# Autodesk Inventor assembly: CONVEYOR-02
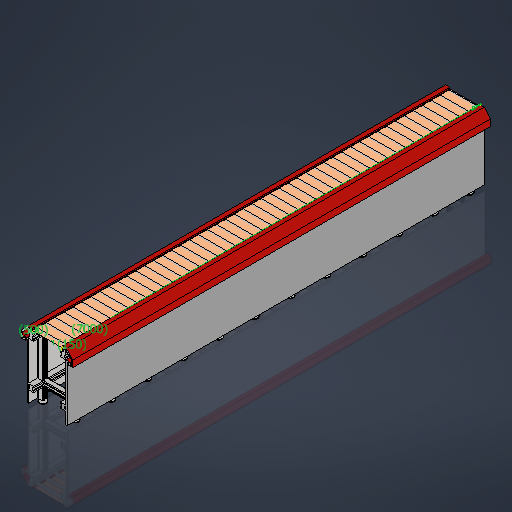
[picture p0: Inventor's stored thumbnail of the model, 512x512]
Saved by Autodesk Inventor 2025 (Build 290162000, 162)
## iProperties
RuleStatus: InUse
Created: 2024-05-06
Part Number: CONVEYOR-02
Document SubType Name: Assembly
Designer: zulet
rollerSeparation: 150,000 mm
conveyorLength: 7000,000 mm
rollerLength: 500,000 mm
Author: zulet
## Documents named in this file (8)
- D:\UNAL\2024-1S\APM\Digital Factory\Conveyor System\CONVEYOR\CONVEYOR-500x7000x1140.iam
- D:\UNAL\2024-1S\APM\Digital Factory\Conveyor System\CONVEYOR STRUCTURE.ipt
- D:\UNAL\2024-1S\APM\Digital Factory\Conveyor System\CONVEYOR ROLLER.ipt
- D:\UNAL\2024-1S\APM\Digital Factory\Conveyor System\CONVEYOR SURFACE.ipt
- D:\UNAL\2024-1S\APM\Digital Factory\Conveyor System\CONVEYOR STRUCTURE\CONVEYOR STRUCTURE-02.ipt
- D:\UNAL\2024-1S\APM\Digital Factory\Conveyor System\CONVEYOR ROLLER\CR-500.ipt
- D:\UNAL\2024-1S\APM\Digital Factory\Conveyor System\CONVEYOR SURFACE\CONVEYOR SURFACE-500x7000.ipt
- D:\UNAL\2024-1S\APM\Digital Factory\Conveyor System\CONVEYOR.iam
## Components (49 placed, 3 different names)
1. CONVEYOR STRUCTURE-02:1 — Mate:1, Mate:2, Rigid:1
2. CONVEYOR SURFACE-500x7000:1 — Rigid:1
3. CR-500:1 — Mate:1, Mate:2
4. CR-500:2
5. CR-500:3
6. CR-500:4
7. CR-500:5
8. CR-500:6
9. CR-500:7
10. CR-500:8
11. CR-500:9
12. CR-500:10
13. CR-500:11
14. CR-500:12
15. CR-500:13
16. CR-500:14
17. CR-500:15
18. CR-500:16
19. CR-500:17
20. CR-500:18
21. CR-500:19
22. CR-500:20
23. CR-500:21
24. CR-500:22
25. CR-500:23
26. CR-500:24
27. CR-500:25
28. CR-500:26
29. CR-500:27
30. CR-500:28
31. CR-500:29
32. CR-500:30
33. CR-500:31
34. CR-500:32
35. CR-500:33
36. CR-500:34
37. CR-500:35
38. CR-500:36
39. CR-500:37
40. CR-500:38
41. CR-500:40
42. CR-500:41
43. CR-500:42
44. CR-500:43
45. CR-500:44
46. CR-500:45
47. CR-500:46
48. CR-500:47
49. CR-500:48
## Component patterns: (47 elements, first: CR-500:1)
## Relationships (3: Mate 2, WeldJoint 1)
- Mate:1: CONVEYOR STRUCTURE-02:1 ↔ CR-500:1
- Mate:2: CONVEYOR STRUCTURE-02:1 ↔ CR-500:1
- Rigid:1 [WeldJoint]: CONVEYOR STRUCTURE-02:1 ↔ CONVEYOR SURFACE-500x7000:1
